# Autodesk Inventor assembly: Thumb Nut
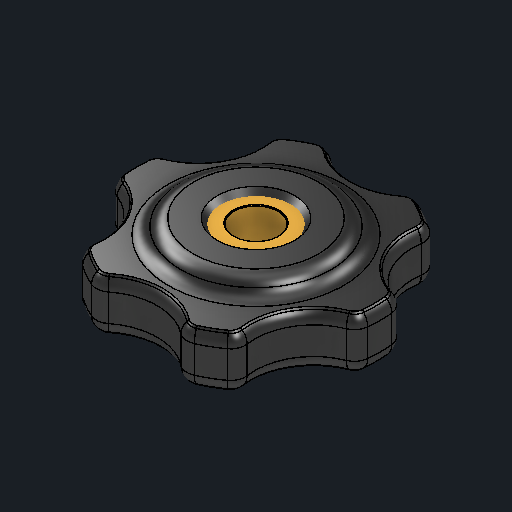
[picture p0: Inventor's stored thumbnail of the model, 512x512]
Saved by Autodesk Inventor 2026.1 (Build 301233020, 233B)
## iProperties
Created: 2025-05-11
Part Number: Thumb Nut
Document SubType Name: Assembly
Designer: Joshua Eah
Author: Joshua Eah
## Documents named in this file (3)
- C:\Users\JoshuaEah\Documents\GitHub\Voron-0\CAD\Z Axis\Subassemblies\Thumb Nut.iam
- C:\Users\JoshuaEah\Documents\GitHub\Voron-0\CAD\Z Axis\Parts\Thumb Nut.ipt
- C:\Users\JoshuaEah\Documents\GitHub\Voron-0\CAD\Hardware\M3 Threaded Insert.ipt
## Components (2 placed, 2 different names)
1. Thumb Nut:1 — Insert:1
2. M3 Threaded Insert:1 — Insert:1
## Relationships (1: Insert 1)
- Insert:1: Thumb Nut:1 ↔ M3 Threaded Insert:1
